# Autodesk Inventor assembly: subassembly_jar_jarcone
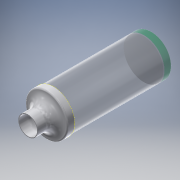
[picture p0: Inventor's stored thumbnail of the model, 180x180]
Saved by Autodesk Inventor 2019 (Build 230136000, 136)
## iProperties
Created: 2019-01-23
Part Number: subassembly_jar_jarcone
Document SubType Name: Assembly
Designer: jmc
Author: jmc
## Documents named in this file (3)
- C:\Users\l0086\Desktop\Models\CatFeeder\version4 (auger)\subassembly_jar_jarcone.iam
- C:\Users\l0086\Desktop\Models\CatFeeder\Jar\Jar.ipt
- C:\Users\l0086\Desktop\Models\CatFeeder\JarCone\version2\cono_nuevo.ipt
## Components (2 placed, 2 different names)
1. Jar:1 — Rigid:2
2. cono_nuevo:1 — Rigid:2
## Relationships (1: WeldJoint 1)
- Rigid:2 [WeldJoint]: Jar:1 ↔ cono_nuevo:1
